# Autodesk Inventor assembly: Chuck Assembly
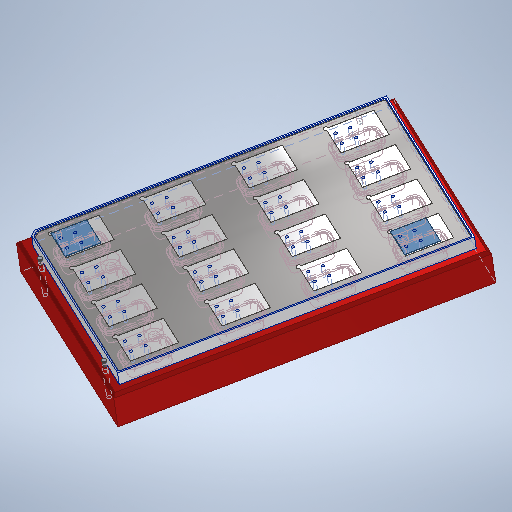
[picture p0: Inventor's stored thumbnail of the model, 512x512]
Saved by Autodesk Inventor 2025 (Build 290162000, 162)
## iProperties
Created: 2021-01-11
Part Number: Chuck Assembly
Document SubType Name: Assembly
Designer: caleb
Author: caleb
## Documents named in this file (5)
- C:\Users\cfang\Desktop\nebraska-silicon-lab\Hardware\ETL\Module Assembly\Chuck - 16-pocket V2\Chuck - 16-pocket - V2.iam
- C:\Users\cfang\Desktop\nebraska-silicon-lab\Hardware\ETL\Module Assembly\Chuck - 16-pocket V2\Chuck - 16-pocket - V2.ipt
- C:\Users\cfang\Desktop\nebraska-silicon-lab\Hardware\ETL\Module Assembly\Chuck - V3\93600A304_316 Stainless Steel Dowel Pin\93600A304_316 Stainless Steel Dowel Pin.ipt
- C:\Users\cfang\Desktop\nebraska-silicon-lab\Hardware\ETL\Module Assembly\BBM Staging Plate - V2\BBM Staging Plate Assembly - V2.iam
- C:\Users\cfang\Desktop\nebraska-silicon-lab\Hardware\ETL\Module Assembly\Chuck - 16-pocket V2\o-ring installed.ipt
## Components (22 placed, 4 different names)
1. Chuck - 16-pocket - V2:1 — Insert:1, Insert:2, Insert:3, Insert:4, Mate:1, Angle:1, Mate:2, Mate:3
2. 93600A304_316 Stainless Steel Dowel Pin:1 — Insert:1, Tangent:2
3. 93600A304_316 Stainless Steel Dowel Pin:2 — Insert:2, Tangent:3
4. 93600A304_316 Stainless Steel Dowel Pin:3 — Insert:3, Tangent:1
5. 93600A304_316 Stainless Steel Dowel Pin:4 — Insert:4
6. BBM Staging Plate Assembly - V2:1 [sub-assembly] — Mate:1, Tangent:1, Tangent:2, Tangent:3, Angle:1
7. o-ring installed:1 — Mate:2, Mate:3
8. o-ring installed:2
9. o-ring installed:3
10. o-ring installed:4
11. o-ring installed:5
12. o-ring installed:6
13. o-ring installed:7
14. o-ring installed:8
15. o-ring installed:9
16. o-ring installed:10
17. o-ring installed:11
18. o-ring installed:12
19. o-ring installed:13
20. o-ring installed:14
21. o-ring installed:15
22. o-ring installed:16
## Component patterns: (16 elements, first: o-ring installed:1)
## Relationships (11: Insert 4, Mate 3, Tangent 3, Angle 1)
- Insert:1 (-5 mm): Chuck - 16-pocket - V2:1 ↔ 93600A304_316 Stainless Steel Dowel Pin:1
- Insert:2 (-5 mm): Chuck - 16-pocket - V2:1 ↔ 93600A304_316 Stainless Steel Dowel Pin:2
- Insert:3 (-5 mm): Chuck - 16-pocket - V2:1 ↔ 93600A304_316 Stainless Steel Dowel Pin:3
- Insert:4 (-5 mm): Chuck - 16-pocket - V2:1 ↔ 93600A304_316 Stainless Steel Dowel Pin:4
- Mate:1: Chuck - 16-pocket - V2:1 ↔ BBM Staging Plate Assembly - V2:1
- Tangent:1: 93600A304_316 Stainless Steel Dowel Pin:3 ↔ BBM Staging Plate Assembly - V2:1
- Tangent:2: 93600A304_316 Stainless Steel Dowel Pin:1 ↔ BBM Staging Plate Assembly - V2:1
- Tangent:3: 93600A304_316 Stainless Steel Dowel Pin:2 ↔ BBM Staging Plate Assembly - V2:1
- Angle:1 (0 deg): Chuck - 16-pocket - V2:1 ↔ BBM Staging Plate Assembly - V2:1
- Mate:2 (1 mm): Chuck - 16-pocket - V2:1 ↔ o-ring installed:1
- Mate:3 (1 mm): Chuck - 16-pocket - V2:1 ↔ o-ring installed:1
